# Autodesk Inventor assembly: Delivery bin outside arm
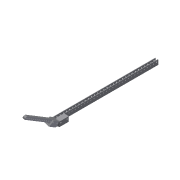
[picture p0: Inventor's stored thumbnail of the model, 180x180]
Saved by Autodesk Inventor 2018 (Build 220112000, 112)
## iProperties
Created: 2019-01-05
Part Number: Delivery bin outside arm
Document SubType Name: Assembly
Designer: ball
Author: ball
## Documents named in this file (4)
- C:\FTC\FTC8863CAD\2018Robot\Delivery bin outside arm.iam
- C:\FTC\FTC8863CAD\Actobotics\585 parts\585399.ipt
- C:\FTC\FTC8863CAD\Actobotics\585 parts\585416.ipt
- C:\FTC\FTC8863CAD\2018Robot\Delivery bin arm connector.ipt
## Components (3 placed, 3 different names)
1. 585399:2 — Mate:1, Mate:2, Mate:3
2. 585416:1 — Mate:4, Mate:5, Mate:6
3. Delivery bin arm connector:1 — Mate:1, Mate:2, Mate:3, Mate:4, Mate:5, Mate:6
## Relationships (6: Mate 6)
- Mate:1: 585399:2 ↔ Delivery bin arm connector:1
- Mate:2: 585399:2 ↔ Delivery bin arm connector:1
- Mate:3: 585399:2 ↔ Delivery bin arm connector:1
- Mate:4: 585416:1 ↔ Delivery bin arm connector:1
- Mate:5: 585416:1 ↔ Delivery bin arm connector:1
- Mate:6: 585416:1 ↔ Delivery bin arm connector:1
